# Autodesk Inventor assembly: Microwave Detection Region v2
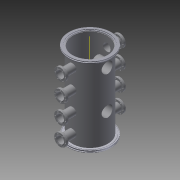
[picture p0: Inventor's stored thumbnail of the model, 180x180]
Saved by Autodesk Inventor 2015 (Build 190159000, 159)
## iProperties
Created: 2014-06-20
Part Number: Microwave Detection Region v2
Document SubType Name: Assembly
Designer: Aki
Author: Aki
## Documents named in this file (4)
- C:\ColdMatter\CADFiles\EDM Machine\Microwave Detection Region\Microwave Detection Region v2.iam
- C:\ColdMatter\CADFiles\EDM Machine\Microwave Detection Region\Detection Region Vacuum Collar v2.ipt
- C:\ColdMatter\CADFiles\EDM Machine\Microwave Detection Region\DN35CF Counter Bored.ipt
- C:\ColdMatter\CADFiles\Generic vacuum components\ISO200SS Bored K Flange.ipt
## Components (11 placed, 3 different names)
1. Detection Region Vacuum Collar v2:1 — Rotational:1, Rotational:2, Rotational:3, Rotational:4, Rotational:7, Rotational:8, Rotational:9, Rotational:10, Rotational:11, Rotational:12
2. DN35CF Counter Bored:1 — Rotational:1
3. DN35CF Counter Bored:2 — Rotational:2
4. DN35CF Counter Bored:3 — Rotational:3
5. DN35CF Counter Bored:4 — Rotational:4
6. DN35CF Counter Bored:5 — Rotational:7
7. DN35CF Counter Bored:6 — Rotational:8
8. DN35CF Counter Bored:7 — Rotational:10
9. DN35CF Counter Bored:8 — Rotational:9
10. ISO200SS Bored K Flange:1 — Rotational:11
11. ISO200SS Bored K Flange:2 — Rotational:12
## Relationships (10: RevoluteJoint 10)
- Rotational:1 [RevoluteJoint]: Detection Region Vacuum Collar v2:1 ↔ DN35CF Counter Bored:1
- Rotational:2 [RevoluteJoint]: Detection Region Vacuum Collar v2:1 ↔ DN35CF Counter Bored:2
- Rotational:3 [RevoluteJoint]: Detection Region Vacuum Collar v2:1 ↔ DN35CF Counter Bored:3
- Rotational:4 [RevoluteJoint]: Detection Region Vacuum Collar v2:1 ↔ DN35CF Counter Bored:4
- Rotational:7 [RevoluteJoint]: Detection Region Vacuum Collar v2:1 ↔ DN35CF Counter Bored:5
- Rotational:8 [RevoluteJoint]: Detection Region Vacuum Collar v2:1 ↔ DN35CF Counter Bored:6
- Rotational:9 [RevoluteJoint]: Detection Region Vacuum Collar v2:1 ↔ DN35CF Counter Bored:8
- Rotational:10 [RevoluteJoint]: Detection Region Vacuum Collar v2:1 ↔ DN35CF Counter Bored:7
- Rotational:11 [RevoluteJoint]: Detection Region Vacuum Collar v2:1 ↔ ISO200SS Bored K Flange:1
- Rotational:12 [RevoluteJoint]: Detection Region Vacuum Collar v2:1 ↔ ISO200SS Bored K Flange:2
